# Autodesk Inventor assembly: McCrea_walle_on_one_chain_walle
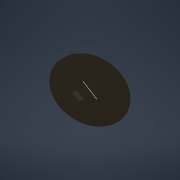
[picture p0: Inventor's stored thumbnail of the model, 180x180]
Saved by Autodesk Inventor 2022 (Build 260153000, 153)
## iProperties
Created: 2022-02-09
Part Number: McCrea_walle_on_one_chain_walle
Document SubType Name: Assembly
Designer: MatusBarany
Author: MatusBarany
## Documents named in this file (4)
- C:\Users\Lukas\Desktop\ard\3D\Walle\FINAL\assembly\McCrea_walle_on_one_chain_walle.iam
- C:\Users\Lukas\Desktop\ard\3D\Walle\FINAL\assembly\McCrea_WALLE_bez_HEAD_walle.iam
- C:\Users\Lukas\Desktop\ard\3D\Walle\FINAL\matus\plocha\McCrea_otočka_walle.ipt
- C:\Users\Lukas\Desktop\ard\3D\Walle\FINAL\matus\plocha\McCrea_ukruhlaPlocha_walle.ipt
## Components (3 placed, 3 different names)
1. McCrea_WALLE_bez_HEAD_walle:1 [sub-assembly] — Mate:1, Flush:1, Flush:2
2. McCrea_otočka_walle:1 — Rotational:1, Angle:1, Mate:1, Flush:1, Flush:2
3. McCrea_ukruhlaPlocha_walle:1 — Rotational:1, Angle:1
## Relationships (5: Flush 2, RevoluteJoint 1, Angle 1, Mate 1)
- Rotational:1 [RevoluteJoint]: McCrea_otočka_walle:1 ↔ McCrea_ukruhlaPlocha_walle:1
- Angle:1 (0 deg): McCrea_otočka_walle:1 ↔ McCrea_ukruhlaPlocha_walle:1
- Mate:1: McCrea_WALLE_bez_HEAD_walle:1 ↔ McCrea_otočka_walle:1
- Flush:1: McCrea_WALLE_bez_HEAD_walle:1 ↔ McCrea_otočka_walle:1
- Flush:2: McCrea_WALLE_bez_HEAD_walle:1 ↔ McCrea_otočka_walle:1
